# Autodesk Inventor assembly: Sestava1
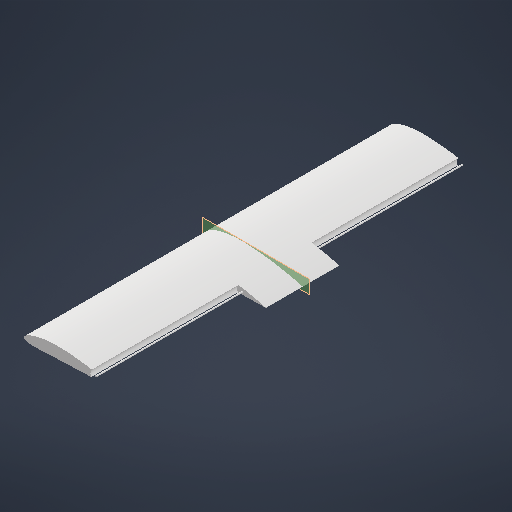
[picture p0: Inventor's stored thumbnail of the model, 512x512]
Saved by Autodesk Inventor 2026 (Build 300175050, 175E)
## iProperties
Created: 2026-01-17
Part Number: Sestava1
Document SubType Name: Assembly
Designer: marti
Author: marti
## Documents named in this file (3)
- F:\Ročníkovka\RP_Svitek\3d model\Sestava1.iam
- F:\Ročníkovka\RP_Svitek\3d model\pokus 1 .ipt
- F:\Ročníkovka\RP_Svitek\3d model\tyč.ipt
## Components (2 placed, 2 different names)
1. pokus 1 :1 — Stejný směr:1, Vložit:1
2. tyč:1 — Vložit:1
## Relationships (2: Flush 1, Insert 1)
- Stejný směr:1 [Flush]: pokus 1 :1
- Vložit:1 [Insert] (-300 mm): pokus 1 :1 ↔ tyč:1
